# Autodesk Inventor assembly: vertical_mirrored
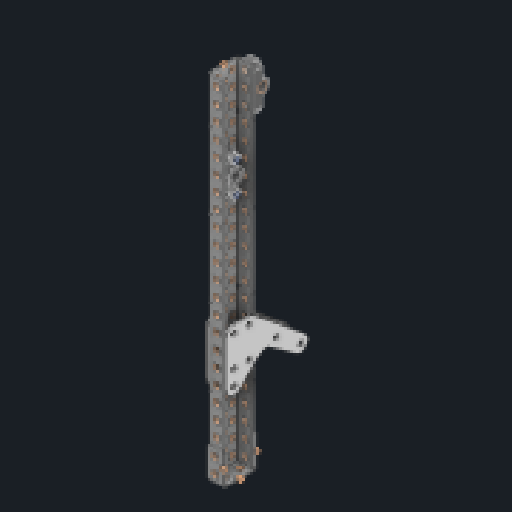
[picture p0: Inventor's stored thumbnail of the model, 512x512]
Saved by Autodesk Inventor 2025 (Build 290162000, 162)
## iProperties
Created: 2024-10-13
Part Number: vertical_mirrored
Document SubType Name: Assembly
Designer: Averey Ku
Author: Averey Ku
## Documents named in this file (10)
- D:\vex_robotics_high_stakes\hardware\cad\bots\high_stakes_v2\tower\structure\side_mirrored\vertical_mirrored.iam
- D:\vex_robotics_high_stakes\hardware\cad\bots\high_stakes_v2\tower\structure\side_mirrored\Alu C 2x2x2x1_mirrored.ipt
- D:\vex_robotics_high_stakes\hardware\cad\bots\high_stakes_v2\tower\structure\side_mirrored\Alu C 1x2x1x23_mirrored.ipt
- D:\vex_robotics_high_stakes\hardware\cad\bots\high_stakes_v2\tower\structure\side_mirrored\HS Pillow Bearing Block_mirrored.ipt
- D:\vex_robotics_high_stakes\hardware\cad\bots\high_stakes_v2\tower\structure\side_mirrored\triangle_brace_gusset_mirrored.ipt
- D:\vex_robotics_high_stakes\hardware\cad\robpros_cad_lib\Motion\Shaft HS\HS Bearing Flat.ipt
- D:\vex_robotics_high_stakes\hardware\cad\VEX-CAD-Inventor\Structure\Hardware\Screw Shoulder Robosource\SScrew Shoulder Smooth .500 x .04.ipt
- D:\vex_robotics_high_stakes\hardware\cad\VEX-CAD-Inventor\Structure\Hardware\Screw Shoulder Robosource.ipt
- D:\vex_robotics_high_stakes\hardware\cad\VEX-CAD-Inventor\Structure\Hardware\Nut Nylon\Nut Nylon - White.ipt
- D:\vex_robotics_high_stakes\hardware\cad\VEX-CAD-Inventor\Structure\Hardware\Nut Nylon.ipt
## Components (10 placed, 7 different names)
1. Alu C 2x2x2x1_mirrored:1 — Mate:2, Insert:1, Mate:1
2. Alu C 1x2x1x23_mirrored:1 — Insert:1, Mate:1, Mate:5, Insert:4, Mate:7, Insert:6, Mate:8, Insert:7, Insert:7, Mate:8, Insert:8, Insert:9
3. HS Pillow Bearing Block_mirrored:1 — Mate:5, Insert:4
4. triangle_brace_gusset_mirrored:1 — Mate:7, Insert:6
5. triangle_brace_gusset_mirrored:2 — Mate:8, Insert:7
6. HS Bearing Flat:1 — Insert:7, Mate:8
7. SScrew Shoulder Smooth .500 x .04:1 — Insert:8
8. Nut Nylon - White:1
9. SScrew Shoulder Smooth .500 x .04:2 — Insert:9
10. Nut Nylon - White:2
## Relationships (17: Insert 9, Mate 8)
- Mate:2: Alu C 2x2x2x1_mirrored:1
- Insert:1: Alu C 2x2x2x1_mirrored:1 ↔ Alu C 1x2x1x23_mirrored:1
- Mate:1: Alu C 2x2x2x1_mirrored:1 ↔ Alu C 1x2x1x23_mirrored:1
- Mate:5: Alu C 1x2x1x23_mirrored:1 ↔ HS Pillow Bearing Block_mirrored:1
- Insert:4: Alu C 1x2x1x23_mirrored:1 ↔ HS Pillow Bearing Block_mirrored:1
- Mate:7: Alu C 1x2x1x23_mirrored:1 ↔ triangle_brace_gusset_mirrored:1
- Insert:6: Alu C 1x2x1x23_mirrored:1 ↔ triangle_brace_gusset_mirrored:1
- Mate:8: Alu C 1x2x1x23_mirrored:1 ↔ triangle_brace_gusset_mirrored:2
- Insert:7 (12.7 mm): Alu C 1x2x1x23_mirrored:1 ↔ triangle_brace_gusset_mirrored:2
- [Mate]: SScrew Shoulder Smooth .500 x .04:1 ↔ Nut Nylon - White:1
- [Insert]: HS Bearing Flat:1 ↔ Nut Nylon - White:1
- [Mate]: SScrew Shoulder Smooth .500 x .04:2 ↔ Nut Nylon - White:2
- [Insert]: HS Bearing Flat:1 ↔ Nut Nylon - White:2
- Insert:7: Alu C 1x2x1x23_mirrored:1 ↔ HS Bearing Flat:1
- Mate:8: Alu C 1x2x1x23_mirrored:1 ↔ HS Bearing Flat:1
- Insert:8: Alu C 1x2x1x23_mirrored:1 ↔ SScrew Shoulder Smooth .500 x .04:1
- Insert:9: Alu C 1x2x1x23_mirrored:1 ↔ SScrew Shoulder Smooth .500 x .04:2
## Named parameters: d12_d3 = 0 mm, d15_d12_d3 = 0 mm
